# Autodesk Inventor assembly: Luftkissenboot
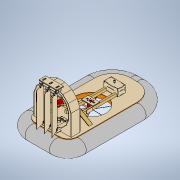
[picture p0: Inventor's stored thumbnail of the model, 180x180]
Saved by Autodesk Inventor 2020.3 (Build 243373000, 373)
## iProperties
Company: HTBLuVA St. Pölten
Created: 2020-02-10
Part Number: Luftkissenboot
Document SubType Name: Assembly
Designer: Stefan Deimel
Mass: 445608 g
Surface Area: 116837 cm^2
Volume: 445608 cm^3
Density: 1 g/cm^3
Project: Diplomarbeit
Description: Luftkissenboot
Author: Stefan
Title: Luftkissenboot
Subject: Diplomarbeit
Revision Number: 3.1
## Documents named in this file (8)
- D:\Stefan\Schule\HTL\Diplomarbeit\git\Inventor\Luftkissenboot.iam
- D:\Stefan\Schule\HTL\Diplomarbeit\git\Inventor\Schlauchoot.ipt
- D:\Stefan\Schule\HTL\Diplomarbeit\git\Inventor\Motor.ipt
- D:\Stefan\Schule\HTL\Diplomarbeit\git\Inventor\Propeller.ipt
- D:\Stefan\Schule\HTL\Diplomarbeit\git\Inventor\Lenker\Lenkung.iam
- D:\Stefan\Schule\HTL\Diplomarbeit\git\Inventor\Bodenplatte\Bodenplatte.iam
- C:\Users\Stefan\Documents\Inventor\Content Center Files\R2020\de-DE\ISO 4016\ISO 4016 - M6 x 30.ipt
- D:\Stefan\Schule\HTL\Diplomarbeit\git\Inventor\hintererAufbau\hintererAufbau.iam
## Components (13 placed, 7 different names)
1. Schlauchoot:1
2. Motor:2 — Drehbar:27, Passend:8, Passend:9, Passend:10
3. Propeller:1 — Drehbar:26, Drehbar:27
4. Propeller:2 — Drehbar:26
5. Motor:3 — Drehbar:23, Passend:11, Passend:12, Passend:13
6. Propeller:5 — Drehbar:23
7. Lenkung:1 [sub-assembly] — Passend:5, Passend:7, Fluchtend:1
8. Bodenplatte:1 [sub-assembly] — Einfügen:88, Einfügen:89, Einfügen:90, Einfügen:91, Passend:5, Passend:6, Passend:7, Passend:8, Passend:9, Passend:10, Fluchtend:1, Fluchtend:2, Fluchtend:3
9. ISO 4016 M6 x 30:1 — Einfügen:88
10. ISO 4016 M6 x 30:2 — Einfügen:89
11. ISO 4016 M6 x 30:3 — Einfügen:90
12. ISO 4016 M6 x 30:4 — Einfügen:91
13. hintererAufbau:1 [sub-assembly] — Passend:6, Passend:11, Passend:12, Passend:13, Fluchtend:2, Fluchtend:3
## Relationships (19: Mate 9, Insert 4, RevoluteJoint 3, Flush 3)
- Drehbar:23 [RevoluteJoint] (15 mm): Motor:3 ↔ Propeller:5
- Drehbar:26 [RevoluteJoint]: Propeller:1 ↔ Propeller:2
- Drehbar:27 [RevoluteJoint]: Motor:2 ↔ Propeller:1
- Einfügen:88 [Insert]: Bodenplatte:1 ↔ ISO 4016 M6 x 30:1
- Einfügen:89 [Insert]: Bodenplatte:1 ↔ ISO 4016 M6 x 30:2
- Einfügen:90 [Insert]: Bodenplatte:1 ↔ ISO 4016 M6 x 30:3
- Einfügen:91 [Insert]: Bodenplatte:1 ↔ ISO 4016 M6 x 30:4
- Passend:5 [Mate]: Lenkung:1 ↔ Bodenplatte:1
- Passend:6 [Mate]: Bodenplatte:1 ↔ hintererAufbau:1
- Passend:7 [Mate] (5 mm): Lenkung:1 ↔ Bodenplatte:1
- Passend:8 [Mate]: Motor:2 ↔ Bodenplatte:1
- Passend:9 [Mate]: Motor:2 ↔ Bodenplatte:1
- Passend:10 [Mate] (1 mm): Motor:2 ↔ Bodenplatte:1
- Passend:11 [Mate]: Motor:3 ↔ hintererAufbau:1
- Passend:12 [Mate]: Motor:3 ↔ hintererAufbau:1
- Passend:13 [Mate] (0.5 mm): Motor:3 ↔ hintererAufbau:1
- Fluchtend:1 [Flush] (315 mm): Lenkung:1 ↔ Bodenplatte:1
- Fluchtend:2 [Flush] (15 mm): Bodenplatte:1 ↔ hintererAufbau:1
- Fluchtend:3 [Flush] (55 mm): Bodenplatte:1 ↔ hintererAufbau:1
